# Autodesk Inventor assembly: Plate Assembly
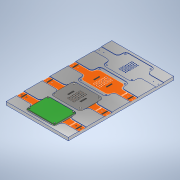
[picture p0: Inventor's stored thumbnail of the model, 180x180]
Saved by Autodesk Inventor 2022 (Build 260153000, 153)
## iProperties
Created: 2021-07-16
Part Number: Plate Assembly
Document SubType Name: Assembly
Designer: Caleb
Author: Caleb
## Documents named in this file (7)
- C:\Users\Caleb\Desktop\nebraska-silicon-lab\Hardware\ETL\Module Assembly\Tamale Assembly Plate\Plate Assembly.iam
- C:\Users\Caleb\Desktop\nebraska-silicon-lab\Hardware\ETL\Module Assembly\Tamale Assembly Plate\Tamale Assembly Plate.ipt
- C:\Users\Caleb\Desktop\nebraska-silicon-lab\Hardware\ETL\Module Assembly\Tamale Assembly Plate\Flex Assembly.iam
- C:\Users\Caleb\Desktop\nebraska-silicon-lab\Hardware\ETL\Module Assembly\Tamale Assembly Plate\spacer.ipt
- C:\Users\Caleb\Desktop\nebraska-silicon-lab\Hardware\ETL\Module Assembly\Tamale Assembly Plate\90910A443_BUTTON HEAD TORX SCREWS.ipt
- C:\Users\Caleb\Desktop\nebraska-silicon-lab\Hardware\ETL\Module Assembly\Tamale Assembly Plate\Mock Module PCB.iam
- C:\Users\Caleb\Desktop\nebraska-silicon-lab\Hardware\ETL\Module Assembly\Tamale Assembly Plate\91585A353_18-8 STAINLESS STEEL DOWEL PIN.ipt
## Components (19 placed, 6 different names)
1. Tamale Assembly Plate:1 — Mate:1, Mate:2, Mate:3, Flush:1, Flush:2, Flush:3, Mate:6, Mate:7, Insert:1, Mate:10, Mate:11, Insert:7, Insert:12, Insert:13, Insert:14, Insert:15, Insert:16, Insert:17, Insert:18, Insert:19, Insert:20
2. Flex Assembly:1 [sub-assembly] — Mate:2, Flush:2, Mate:9, Insert:7
3. Flex Assembly:2 [sub-assembly] — Mate:3, Flush:3, Insert:20
4. Flex Assembly:4 [sub-assembly] — Mate:1, Flush:1, Mate:5, Insert:1, Insert:2, Insert:3, Insert:4, Insert:5
5. spacer:1 — Mate:5, Mate:6, Mate:7, Mate:8, Angle:1, Insert:6
6. 90910A443_BUTTON HEAD TORX SCREWS:1 — Insert:2
7. 90910A443_BUTTON HEAD TORX SCREWS:2 — Insert:3
8. 90910A443_BUTTON HEAD TORX SCREWS:3 — Insert:5
9. 90910A443_BUTTON HEAD TORX SCREWS:4 — Insert:4
10. Mock Module PCB:1 [sub-assembly] — Mate:8, Angle:1, Insert:6
11. spacer:2 — Mate:9, Mate:10, Mate:11
12. 91585A353_18-8 STAINLESS STEEL DOWEL PIN:1 — Insert:12
13. 91585A353_18-8 STAINLESS STEEL DOWEL PIN:2 — Insert:13
14. 91585A353_18-8 STAINLESS STEEL DOWEL PIN:3 — Insert:14
15. 91585A353_18-8 STAINLESS STEEL DOWEL PIN:4 — Insert:15
16. 91585A353_18-8 STAINLESS STEEL DOWEL PIN:5 — Insert:16
17. 91585A353_18-8 STAINLESS STEEL DOWEL PIN:6 — Insert:17
18. 91585A353_18-8 STAINLESS STEEL DOWEL PIN:7 — Insert:18
19. 91585A353_18-8 STAINLESS STEEL DOWEL PIN:8 — Insert:19
## Relationships (30: Insert 16, Mate 10, Flush 3, Angle 1)
- Mate:1: Tamale Assembly Plate:1 ↔ Flex Assembly:4
- Mate:2: Tamale Assembly Plate:1 ↔ Flex Assembly:1
- Mate:3: Tamale Assembly Plate:1 ↔ Flex Assembly:2
- Flush:1: Tamale Assembly Plate:1 ↔ Flex Assembly:4
- Flush:2: Tamale Assembly Plate:1 ↔ Flex Assembly:1
- Flush:3: Tamale Assembly Plate:1 ↔ Flex Assembly:2
- Mate:5: Flex Assembly:4 ↔ spacer:1
- Mate:6: Tamale Assembly Plate:1 ↔ spacer:1
- Mate:7: Tamale Assembly Plate:1 ↔ spacer:1
- Insert:1: Tamale Assembly Plate:1 ↔ Flex Assembly:4
- Insert:2: Flex Assembly:4 ↔ 90910A443_BUTTON HEAD TORX SCREWS:1
- Insert:3: Flex Assembly:4 ↔ 90910A443_BUTTON HEAD TORX SCREWS:2
- Insert:4: Flex Assembly:4 ↔ 90910A443_BUTTON HEAD TORX SCREWS:4
- Insert:5: Flex Assembly:4 ↔ 90910A443_BUTTON HEAD TORX SCREWS:3
- Mate:8: spacer:1 ↔ Mock Module PCB:1
- Angle:1 (0 deg): spacer:1 ↔ Mock Module PCB:1
- Insert:6: spacer:1 ↔ Mock Module PCB:1
- Mate:9: Flex Assembly:1 ↔ spacer:2
- Mate:10: Tamale Assembly Plate:1 ↔ spacer:2
- Mate:11: Tamale Assembly Plate:1 ↔ spacer:2
- Insert:7: Tamale Assembly Plate:1 ↔ Flex Assembly:1
- Insert:12: Tamale Assembly Plate:1 ↔ 91585A353_18-8 STAINLESS STEEL DOWEL PIN:1
- Insert:13: Tamale Assembly Plate:1 ↔ 91585A353_18-8 STAINLESS STEEL DOWEL PIN:2
- Insert:14: Tamale Assembly Plate:1 ↔ 91585A353_18-8 STAINLESS STEEL DOWEL PIN:3
- Insert:15: Tamale Assembly Plate:1 ↔ 91585A353_18-8 STAINLESS STEEL DOWEL PIN:4
- Insert:16: Tamale Assembly Plate:1 ↔ 91585A353_18-8 STAINLESS STEEL DOWEL PIN:5
- Insert:17: Tamale Assembly Plate:1 ↔ 91585A353_18-8 STAINLESS STEEL DOWEL PIN:6
- Insert:18: Tamale Assembly Plate:1 ↔ 91585A353_18-8 STAINLESS STEEL DOWEL PIN:7
- Insert:19: Tamale Assembly Plate:1 ↔ 91585A353_18-8 STAINLESS STEEL DOWEL PIN:8
- Insert:20: Tamale Assembly Plate:1 ↔ Flex Assembly:2
